# Autodesk Inventor assembly: Motor Mount with Motor
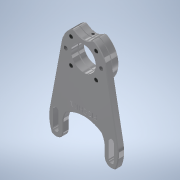
[picture p0: Inventor's stored thumbnail of the model, 180x180]
Saved by Autodesk Inventor 2020.1 (Build 241239000, 239)
## iProperties
Created: 2019-03-01
Part Number: Motor Mount with Motor
Document SubType Name: Assembly
Designer: Petar
Mass: 37.7633 g
Surface Area: 102.459 cm^2
Volume: 12.7696 cm^3
Density: 2.95729 g/cm^3
Author: Petar
## Documents named in this file (7)
- D:\OMG\E-Board\CAD\Inventor\Mechanical Components\Assemblies\Motor Mount - 225 - ALUMINIUM.iam
- D:\OMG\E-Board\CAD\Inventor\Mechanical Components\Motor Mount\Ring Mount\Mount Ring - ALUMINIUM.ipt
- D:\OMG\E-Board\CAD\Inventor\Mechanical Components\Motor Mount\Holder Mount\Motor Holder v3 - 225 - ALUMINIUM.ipt
- D:\OMG\E-Board\CAD\Inventor\Mechanical Components\Assemblies\Motor Mount - 225 - ALUMINIUM\Design Accelerator\Bolted Connection1.iam
- D:\OMG\E-Board\CAD\Inventor\Mechanical Components\Assemblies\Motor Mount - 225 - ALUMINIUM\Design Accelerator\Bolted Connection2.iam
- D:\OMG\E-Board\CAD\Inventor\Mechanical Components\Assemblies\Motor Mount - 225 - ALUMINIUM\Design Accelerator\Bolted Connection3.iam
- D:\OMG\E-Board\CAD\Inventor\Mechanical Components\Assemblies\Motor Mount - 225 - ALUMINIUM\Design Accelerator\Bolted Connection4.iam
## Components (6 placed, 3 different names)
1. Motor Holder v3 - 225 - ALUMINIUM:1 — Rigid:2, Mate:9
2. Mount Ring - ALUMINIUM:1 — Rigid:2, Mate:1, Mate:2, Mate:3, Mate:4, Mate:5, Mate:6, Mate:7, Mate:8, Mate:10
3. Bolted Connection:1 [sub-assembly] — Mate:1, Mate:2
4. Bolted Connection:2 [sub-assembly] — Mate:3, Mate:4
5. Bolted Connection:3 [sub-assembly] — Mate:5, Mate:6
6. Bolted Connection:4 [sub-assembly] — Mate:7, Mate:8
## Relationships (12: Mate 10, WeldJoint 1, Angle 1)
- Rigid:2 [WeldJoint]: Motor Holder v3 - 225 - ALUMINIUM:1 ↔ Mount Ring - ALUMINIUM:1
- Mate:1: Mount Ring - ALUMINIUM:1 ↔ Bolted Connection:1
- Mate:2: Mount Ring - ALUMINIUM:1 ↔ Bolted Connection:1
- Mate:3: Mount Ring - ALUMINIUM:1 ↔ Bolted Connection:2
- Mate:4: Mount Ring - ALUMINIUM:1 ↔ Bolted Connection:2
- Mate:5: Mount Ring - ALUMINIUM:1 ↔ Bolted Connection:3
- Mate:6: Mount Ring - ALUMINIUM:1 ↔ Bolted Connection:3
- Mate:7: Mount Ring - ALUMINIUM:1 ↔ Bolted Connection:4
- Mate:8: Mount Ring - ALUMINIUM:1 ↔ Bolted Connection:4
- Mate:9: Motor Holder v3 - 225 - ALUMINIUM:1
- Angle:1 (0 deg)
- Mate:10: Mount Ring - ALUMINIUM:1
